# Autodesk Inventor assembly: Schrittkette_4_Step
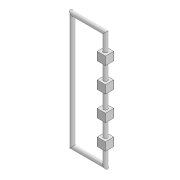
[picture p0: Inventor's stored thumbnail of the model, 180x180]
Saved by Autodesk Inventor 2020 (Build 240168000, 168)
## iProperties
Created: 2020-03-08
Part Number: Schrittkette_4_Step
Document SubType Name: Assembly
Designer: franz
Author: franz
## Documents named in this file (9)
- E:\Privat\Projekte\SPS_Training\Unity_SPS_Simulation\Unity_SPS_Schrittkette\CAD\Schrittkette_4_Step\Schrittkette_4_Step.iam
- E:\Privat\Projekte\SPS_Training\Unity_SPS_Simulation\Unity_SPS_Schrittkette\CAD\Schrittkette_4_Step\Init_Step.ipt
- E:\Privat\Projekte\SPS_Training\Unity_SPS_Simulation\Unity_SPS_Schrittkette\CAD\Schrittkette_4_Step\1_Step.ipt
- E:\Privat\Projekte\SPS_Training\Unity_SPS_Simulation\Unity_SPS_Schrittkette\CAD\Schrittkette_4_Step\2_Step.ipt
- E:\Privat\Projekte\SPS_Training\Unity_SPS_Simulation\Unity_SPS_Schrittkette\CAD\Schrittkette_4_Step\3_Step.ipt
- E:\Privat\Projekte\SPS_Training\Unity_SPS_Simulation\Unity_SPS_Schrittkette\CAD\Schrittkette_4_Step\Transition_Init_1.ipt
- E:\Privat\Projekte\SPS_Training\Unity_SPS_Simulation\Unity_SPS_Schrittkette\CAD\Schrittkette_4_Step\Transition_1_2.ipt
- E:\Privat\Projekte\SPS_Training\Unity_SPS_Simulation\Unity_SPS_Schrittkette\CAD\Schrittkette_4_Step\Transition_2_3.ipt
- E:\Privat\Projekte\SPS_Training\Unity_SPS_Simulation\Unity_SPS_Schrittkette\CAD\Schrittkette_4_Step\Transition_3_Init.ipt
## Components (8 placed, 8 different names)
1. Init_Step:1 — Starr:1
2. 1_Step:1 — Starr:2, Starr:3
3. 2_Step:1 — Starr:4, Starr:5
4. 3_Step:1 — Starr:6, Starr:7
5. Transition_Init_1:1 — Starr:1, Starr:2
6. Transition_1_2:1 — Starr:3, Starr:4
7. Transition_2_3:1 — Starr:5, Starr:6
8. Transition_3_Init:1 — Starr:7
## Relationships (7: WeldJoint 7)
- Starr:1 [WeldJoint]: Init_Step:1 ↔ Transition_Init_1:1
- Starr:2 [WeldJoint]: 1_Step:1 ↔ Transition_Init_1:1
- Starr:3 [WeldJoint]: 1_Step:1 ↔ Transition_1_2:1
- Starr:4 [WeldJoint]: 2_Step:1 ↔ Transition_1_2:1
- Starr:5 [WeldJoint]: 2_Step:1 ↔ Transition_2_3:1
- Starr:6 [WeldJoint]: 3_Step:1 ↔ Transition_2_3:1
- Starr:7 [WeldJoint]: 3_Step:1 ↔ Transition_3_Init:1
## Named parameters: Transitionsdicke = 0.3 mm
